# Autodesk Inventor assembly: Tarea 3 Ensamble Lab dinamica Fabian Aragon
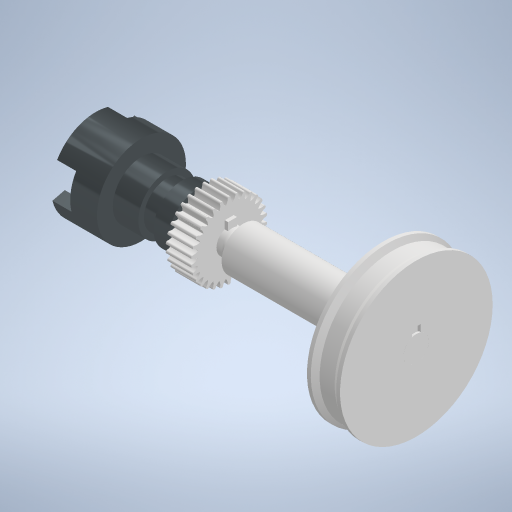
[picture p0: Inventor's stored thumbnail of the model, 512x512]
Saved by Autodesk Inventor 2024 (Build 280153000, 153)
## iProperties
Created: 2024-03-07
Part Number: Tarea 3 Ensamble Lab dinamica Fabian Aragon
Document SubType Name: Assembly
Designer: FabAr
Author: FabAr
## Documents named in this file (6)
- C:\Users\FabAr\OneDrive\Documents\Fabian\Dinamica lab\Tarea 3 Ensamble Lab dinamica Fabian Aragon.iam
- C:\Users\FabAr\Downloads\POLEA.ipt
- C:\Users\FabAr\Downloads\ENGRANE.ipt
- C:\Users\FabAr\Downloads\EJE_CUÑEROS.ipt
- C:\Users\FabAr\Downloads\CUÑA.ipt
- C:\Users\FabAr\Downloads\tarea 3 dinamica.ipt
## Components (6 placed, 5 different names)
1. POLEA:1 — Rigid:1
2. ENGRANE:1 — Cylindrical:1, Flush:1
3. EJE_CUÑEROS:1 — Rigid:1, Cylindrical:1, Flush:1, Planar:1, Mate:1, Mate:2, Planar:2, Mate:3, Mate:4, Rigid:2
4. CUÑA:1 — Planar:1, Mate:1, Mate:2
5. tarea 3 dinamica:1 — Rigid:2
6. CUÑA:2 — Planar:2, Mate:3, Mate:4
## Relationships (10: Mate 4, WeldJoint 2, PlanarJoint 2, CylindricalJoint 1, Flush 1)
- Rigid:1 [WeldJoint]: POLEA:1 ↔ EJE_CUÑEROS:1
- Cylindrical:1: ENGRANE:1 ↔ EJE_CUÑEROS:1
- Flush:1 (5 mm): ENGRANE:1 ↔ EJE_CUÑEROS:1
- Planar:1: EJE_CUÑEROS:1 ↔ CUÑA:1
- Mate:1: EJE_CUÑEROS:1 ↔ CUÑA:1
- Mate:2: EJE_CUÑEROS:1 ↔ CUÑA:1
- Planar:2: EJE_CUÑEROS:1 ↔ CUÑA:2
- Mate:3: EJE_CUÑEROS:1 ↔ CUÑA:2
- Mate:4: EJE_CUÑEROS:1 ↔ CUÑA:2
- Rigid:2 [WeldJoint]: EJE_CUÑEROS:1 ↔ tarea 3 dinamica:1
